# Autodesk Inventor assembly: 后底盘组
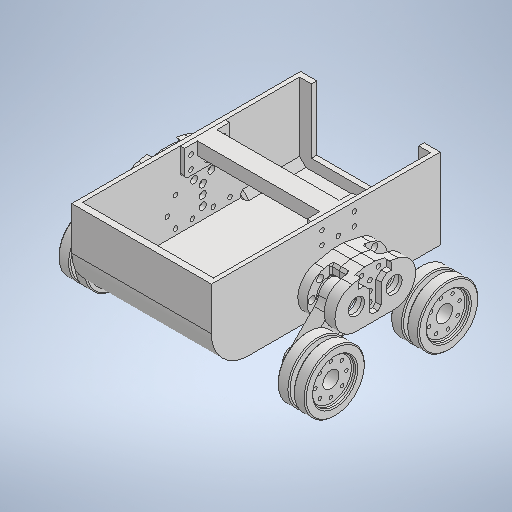
[picture p0: Inventor's stored thumbnail of the model, 512x512]
Saved by Autodesk Inventor 2025.1 (Build 291241000, 241)
## iProperties
Created: 2025-08-27
Part Number: 后底盘组
Document SubType Name: Assembly
Designer: Piw
Author: Piw
## Documents named in this file (4)
- C:\Users\22982\Desktop\急急急\Classis\后底盘组.iam
- C:\Users\22982\Desktop\急急急\Classis\后车架.ipt
- C:\Users\22982\Desktop\急急急\Classis\悬架.iam
- C:\Users\22982\Desktop\急急急\Classis\加强梁.ipt
## Components (4 placed, 3 different names)
1. 后车架:1 — 配合:1, 配合:2, 配合:3, 配合:4, 配合:5, 配合:6, 配合:7, 配合:8, 配合:9
2. 悬架:1 [sub-assembly] — 配合:1, 配合:2, 配合:3
3. 悬架:2 [sub-assembly] — 配合:4, 配合:5, 配合:6
4. 加强梁:1 — 配合:7, 配合:8, 配合:9
## Relationships (9: Mate 9)
- 配合:1 [Mate]: 后车架:1 ↔ 悬架:1
- 配合:2 [Mate]: 后车架:1 ↔ 悬架:1
- 配合:3 [Mate]: 后车架:1 ↔ 悬架:1
- 配合:4 [Mate]: 后车架:1 ↔ 悬架:2
- 配合:5 [Mate]: 后车架:1 ↔ 悬架:2
- 配合:6 [Mate]: 后车架:1 ↔ 悬架:2
- 配合:7 [Mate]: 后车架:1 ↔ 加强梁:1
- 配合:8 [Mate]: 后车架:1 ↔ 加强梁:1
- 配合:9 [Mate]: 后车架:1 ↔ 加强梁:1
